# Autodesk Inventor assembly: Impeller Assembly
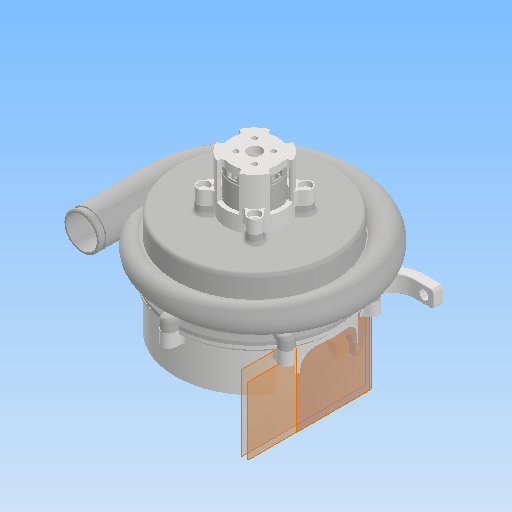
[picture p0: Inventor's stored thumbnail of the model, 512x512]
Saved by Autodesk Inventor 2020 (Build 240168000, 168)
## iProperties
Created: 2020-04-09
Part Number: Impeller Assembly
Document SubType Name: Assembly
Designer: John K
Author: John K
## Documents named in this file (8)
- D:\GrabCAD\MTL Ventilator Design\Breeze V2\Impeller Assembly\Impeller Assembly.iam
- D:\GrabCAD\MTL Ventilator Design\Breeze V2\Impeller Assembly\Turbine housing solid.ipt
- D:\GrabCAD\MTL Ventilator Design\Breeze V2\Impeller Assembly\BRZ-P201.ipt
- D:\GrabCAD\MTL Ventilator Design\Breeze V2\Impeller Assembly\BRZ-P203.ipt
- D:\GrabCAD\MTL Ventilator Design\Breeze V2\Impeller Assembly\Commercial Parts\McMaster\Bushing Flanged Nylon 6389K234.ipt
- D:\GrabCAD\MTL Ventilator Design\Breeze V2\Impeller Assembly\Commercial Parts\McMaster\Shaft Seal 9562K420.ipt
- D:\GrabCAD\MTL Ventilator Design\Breeze V2\Impeller Assembly\Motor Mount.ipt
- D:\GrabCAD\MTL Ventilator Design\Breeze V2\Impeller Assembly\Commercial Parts\Motor\Brushless Motor 2212 2450kv.iam
## Components (7 placed, 7 different names)
1. Turbine housing solid:1 — Mate:1, Mate:2, Mate:3, Mate:5, Insert:1, Mate:6, Mate:7, Mate:8
2. BRZ-P201:1 — Mate:1, Mate:2
3. BRZ-P203:1 — Mate:3, Mate:5, Mate:8
4. Bushing Flanged Nylon 6389K234:1 — Insert:1, Insert:2
5. Shaft Seal 9562K420:1 — Insert:2
6. Motor Mount:1 — Flush:1, Mate:6, Mate:7, Mate:9, Mate:10, Mate:11
7. Brushless Motor 2212 2450kv:1 [sub-assembly] — Mate:9, Mate:10, Mate:11
## Relationships (13: Mate 10, Insert 2, Flush 1)
- Mate:1: Turbine housing solid:1 ↔ BRZ-P201:1
- Mate:2 (-2.5 mm): Turbine housing solid:1 ↔ BRZ-P201:1
- Mate:3: Turbine housing solid:1 ↔ BRZ-P203:1
- Mate:5: Turbine housing solid:1 ↔ BRZ-P203:1
- Insert:1: Turbine housing solid:1 ↔ Bushing Flanged Nylon 6389K234:1
- Insert:2 (-1 mm): Bushing Flanged Nylon 6389K234:1 ↔ Shaft Seal 9562K420:1
- Flush:1: Motor Mount:1
- Mate:6: Turbine housing solid:1 ↔ Motor Mount:1
- Mate:7: Turbine housing solid:1 ↔ Motor Mount:1
- Mate:8: Turbine housing solid:1 ↔ BRZ-P203:1
- Mate:9: Motor Mount:1 ↔ Brushless Motor 2212 2450kv:1
- Mate:10: Motor Mount:1 ↔ Brushless Motor 2212 2450kv:1
- Mate:11: Motor Mount:1 ↔ Brushless Motor 2212 2450kv:1
